# Autodesk Inventor assembly: XT-6
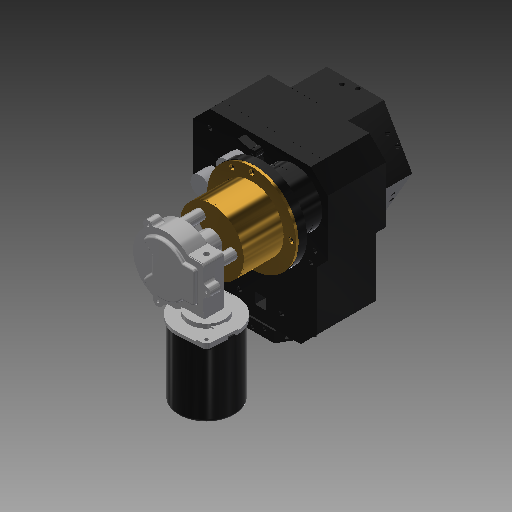
[picture p0: Inventor's stored thumbnail of the model, 512x512]
Saved by Autodesk Inventor 2017 (Build 210142000, 142)
## iProperties
Created: 2019-09-19
Part Number: XT-6
Document SubType Name: Assembly
Designer: Dell
Author: Dell
## Documents named in this file (16)
- C:\Users\Dell\Documents\GitHub\tr2\Actuator 2.0\XT-6.iam
- C:\Users\Dell\Documents\GitHub\tr2\Actuator 2.0\AC01.ipt
- C:\Users\Dell\Documents\GitHub\tr2\Actuator 2.0\AC02.ipt
- C:\Users\Dell\Documents\GitHub\tr2\Actuator 2.0\AC05.ipt
- C:\Users\Dell\Documents\GitHub\tr2\Actuator 2.0\Slewing.iam
- C:\Users\Dell\Documents\GitHub\tr2\Actuator 2.0\Slip Ring.ipt
- C:\Users\Dell\Documents\GitHub\tr2\Actuator 2.0\8mm Mounting Hub.ipt
- C:\Users\Dell\Documents\GitHub\tr2\Actuator 2.0\AEAT-6012.ipt
- C:\Users\Dell\Documents\GitHub\tr2\Actuator 2.0\Series Elastic Gearbox 1.2\Series Elastic Gearbox 1.2.iam
- C:\Users\Dell\Documents\GitHub\tr2\Actuator 2.0\Actuator 2.0\Design Accelerator\Spur Gears3.iam
- C:\Users\Dell\Documents\GitHub\tr2\Actuator 2.0\Actuator 2.0\Design Accelerator\Spur Gears4.iam
- C:\Users\Dell\Documents\GitHub\tr2\Actuator 2.0\Actuator 2.0\Design Accelerator\Spur Gears5.iam
- C:\Users\Dell\Documents\GitHub\tr2\Actuator 2.0\6201-2RS.ipt
- C:\Users\Dell\Documents\GitHub\tr2\Actuator 2.0\AC09.ipt
- C:\Users\Dell\Documents\GitHub\tr2\Actuator 2.0\PN00113-6.iam
- C:\Users\Dell\Documents\GitHub\tr2\Actuator 2.0\AC10.ipt
## Components (17 placed, 13 different names)
1. AC01:1 — Mate:3, Mate:4, Mate:5, Mate:9, Mate:139, Mate:140, Mate:141, Mate:142, Mate:145, Mate:146
2. AC02:1 — Mate:9, Mate:139, Mate:140, Mate:141, Mate:142, Mate:145, Mate:146, Mate:150, Mate:151, Mate:152, Mate:153, Mate:154, Mate:155, Mate:168, Mate:169, Mate:170, Mate:171, Mate:172, Mate:173, Mate:175, Mate:176, Mate:177, Mate:179
3. AC05:1 — Mate:6, Mate:7, Mate:8, Mate:23, Mate:24, Mate:25, Mate:90, Mate:91, Mate:92
4. Slewing:1 [sub-assembly] — Mate:3, Mate:4, Mate:5, Mate:6, Mate:7, Mate:8
5. Slip Ring:2 — Mate:23, Mate:24, Mate:25
6. 8mm Mounting Hub:1 — Mate:119, Mate:148, Mate:173, Mate:174
7. AEAT-6012:1 — Mate:151, Mate:158, Mate:162, Mate:163, Mate:164
8. AEAT-6012:2 — Mate:149, Mate:150, Mate:165, Mate:166, Mate:167
9. Series Elastic Gearbox 1.2:1 [sub-assembly] — Mate:90, Mate:91, Mate:92, Mate:113, Mate:114, Mate:116, Mate:120, Mate:134, Mate:143, Mate:156
10. Spur Gears:1 [sub-assembly] — Mate:113, Mate:114, Mate:116, Mate:119, Mate:120, Rotation:1, Mate:144, Mate:148, Flush:1, Mate:174
11. Spur Gears:2 [sub-assembly] — Mate:134, Mate:143, Mate:144, Mate:156, Mate:158
12. Spur Gears:3 [sub-assembly] — Rotation:1, Mate:149, Flush:1
13. 6201-2RS:1 — Mate:154, Mate:155
14. 6201-2RS:2 — Mate:152, Mate:153
15. AC09:1 — Mate:162, Mate:163, Mate:164, Mate:165, Mate:166, Mate:167, Mate:168, Mate:169, Mate:170, Mate:171, Mate:172
16. PN00113-6:1 [sub-assembly] — Mate:175, Mate:180, Mate:181, Mate:182
17. AC10:1 — Mate:176, Mate:177, Mate:179, Mate:180, Mate:181, Mate:182
## Relationships (59: Mate 57, RelateRotation 1, Flush 1)
- Mate:3: AC01:1 ↔ Slewing:1
- Mate:4: AC01:1 ↔ Slewing:1
- Mate:5: AC01:1 ↔ Slewing:1
- Mate:6: AC05:1 ↔ Slewing:1
- Mate:7: AC05:1 ↔ Slewing:1
- Mate:8: AC05:1 ↔ Slewing:1
- Mate:9: AC01:1 ↔ AC02:1
- Mate:23: AC05:1 ↔ Slip Ring:2
- Mate:24 (5 mm): AC05:1 ↔ Slip Ring:2
- Mate:25: AC05:1 ↔ Slip Ring:2
- Mate:90: AC05:1 ↔ Series Elastic Gearbox 1.2:1
- Mate:91: AC05:1 ↔ Series Elastic Gearbox 1.2:1
- Mate:92: AC05:1 ↔ Series Elastic Gearbox 1.2:1
- Mate:113: Series Elastic Gearbox 1.2:1 ↔ Spur Gears:1
- Mate:114: Series Elastic Gearbox 1.2:1 ↔ Spur Gears:1
- Mate:116: Series Elastic Gearbox 1.2:1 ↔ Spur Gears:1
- Mate:119: 8mm Mounting Hub:1 ↔ Spur Gears:1
- Mate:120: Series Elastic Gearbox 1.2:1 ↔ Spur Gears:1
- Rotation:1 [RelateRotation] (1.0714 ul): Spur Gears:1 ↔ Spur Gears:3
- Mate:134: Series Elastic Gearbox 1.2:1 ↔ Spur Gears:2
- Mate:139: AC01:1 ↔ AC02:1
- Mate:140: AC01:1 ↔ AC02:1
- Mate:141: AC01:1 ↔ AC02:1
- Mate:142: AC01:1 ↔ AC02:1
- Mate:143: Series Elastic Gearbox 1.2:1 ↔ Spur Gears:2
- Mate:144 (1 mm): Spur Gears:1 ↔ Spur Gears:2
- Mate:145: AC01:1 ↔ AC02:1
- Mate:146: AC01:1 ↔ AC02:1
- Mate:148: 8mm Mounting Hub:1 ↔ Spur Gears:1
- Mate:149: AEAT-6012:2 ↔ Spur Gears:3
- Flush:1: Spur Gears:1 ↔ Spur Gears:3
- Mate:150: AC02:1 ↔ AEAT-6012:2
- Mate:151: AC02:1 ↔ AEAT-6012:1
- Mate:152: AC02:1 ↔ 6201-2RS:2
- Mate:153: AC02:1 ↔ 6201-2RS:2
- Mate:154: AC02:1 ↔ 6201-2RS:1
- Mate:155: AC02:1 ↔ 6201-2RS:1
- Mate:156: Series Elastic Gearbox 1.2:1 ↔ Spur Gears:2
- Mate:158: AEAT-6012:1 ↔ Spur Gears:2
- Mate:162: AEAT-6012:1 ↔ AC09:1
- Mate:163: AEAT-6012:1 ↔ AC09:1
- Mate:164: AEAT-6012:1 ↔ AC09:1
- Mate:165: AEAT-6012:2 ↔ AC09:1
- Mate:166: AEAT-6012:2 ↔ AC09:1
- Mate:167: AEAT-6012:2 ↔ AC09:1
- Mate:168: AC02:1 ↔ AC09:1
- Mate:169: AC02:1 ↔ AC09:1
- Mate:170: AC02:1 ↔ AC09:1
- Mate:171: AC02:1 ↔ AC09:1
- Mate:172: AC02:1 ↔ AC09:1
- Mate:173: AC02:1 ↔ 8mm Mounting Hub:1
- Mate:174: 8mm Mounting Hub:1 ↔ Spur Gears:1
- Mate:175: AC02:1 ↔ PN00113-6:1
- Mate:176: AC02:1 ↔ AC10:1
- Mate:177: AC02:1 ↔ AC10:1
- Mate:179: AC02:1 ↔ AC10:1
- Mate:180: PN00113-6:1 ↔ AC10:1
- Mate:181: PN00113-6:1 ↔ AC10:1
- Mate:182: PN00113-6:1 ↔ AC10:1
